# Autodesk Inventor assembly: battery_pack_16s.ipt
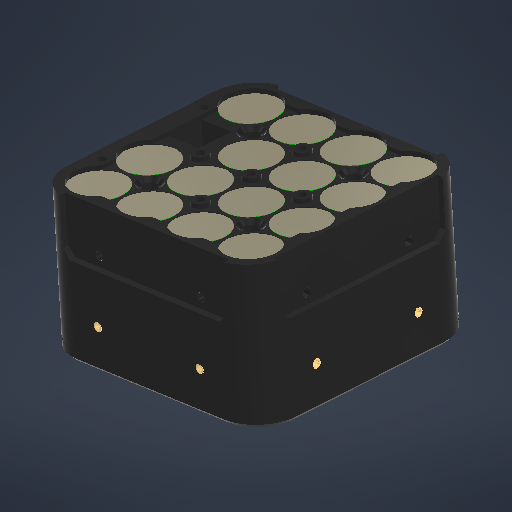
[picture p0: Inventor's stored thumbnail of the model, 512x512]
Saved by Autodesk Inventor 2026.1 (Build 301233000, 233)
## iProperties
Created: 2026-03-12
Part Number: battery_pack_16s.ipt
Document SubType Name: Assembly
Designer: aaron
Author: aaron
## Documents named in this file (6)
- D:\work\loopandpixel\openworkoutsystem\cad\v5\battery_pack_16s.ipt.iam
- D:\work\loopandpixel\openworkoutsystem\cad\v5\battery_26650_lifepo4.ipt
- D:\work\loopandpixel\openworkoutsystem\cad\v5\battery_pack_16s_front.ipt
- D:\work\loopandpixel\openworkoutsystem\cad\v5\battery_pack_cover_rear.ipt
- C:\Users\aaron\OneDrive\Documents\Inventor\Content Center Files\R2026\en-US\IS 6761\IS 6761 - M3 x 8 - 0.5.ipt
- D:\work\loopandpixel\openworkoutsystem\cad\v5\ruthex_RX-M3x5_7\ruthex_RX-M3x5_7\ruthex_RX-M3x5_7.iam
## Components (27 placed, 5 different names)
1. battery_pack_16s_front:1 — Insert:9, Mate:1, Flush:1, Flush:2, Insert:10, Insert:11, Insert:12, Insert:13, Insert:14, Insert:15
2. battery_pack_cover_rear:1 — Mate:1, Flush:1, Flush:2, Mate:2, Mate:3, Mate:4, Mate:5
3. IS 6761 M3 x 8:1 — Mate:2
4. IS 6761 M3 x 8:2 — Mate:3
5. IS 6761 M3 x 8:3 — Mate:4
6. IS 6761 M3 x 8:4 — Mate:5
7. ruthex_RX-M3x5_7:1 [sub-assembly] — Insert:11
8. ruthex_RX-M3x5_7:2 [sub-assembly] — Insert:10
9. ruthex_RX-M3x5_7:3 [sub-assembly] — Insert:12
10. ruthex_RX-M3x5_7:4 [sub-assembly] — Insert:13
11. ruthex_RX-M3x5_7:5 [sub-assembly] — Insert:14
12. ruthex_RX-M3x5_7:6 [sub-assembly] — Insert:15
13. battery_26650_lifepo4:1 — Insert:9
14. battery_26650_lifepo4:2
15. battery_26650_lifepo4:3
16. battery_26650_lifepo4:4
17. battery_26650_lifepo4:5
18. battery_26650_lifepo4:6
19. battery_26650_lifepo4:7
20. battery_26650_lifepo4:8
21. battery_26650_lifepo4:10
22. battery_26650_lifepo4:11
23. battery_26650_lifepo4:12
24. battery_26650_lifepo4:13
25. battery_26650_lifepo4:14
26. battery_26650_lifepo4:15
27. battery_26650_lifepo4:16
## Component patterns: (16 elements, first: battery_26650_lifepo4:1)
## Relationships (14: Insert 7, Mate 5, Flush 2)
- Insert:9: battery_pack_16s_front:1 ↔ battery_26650_lifepo4:1
- Mate:1: battery_pack_16s_front:1 ↔ battery_pack_cover_rear:1
- Flush:1: battery_pack_16s_front:1 ↔ battery_pack_cover_rear:1
- Flush:2: battery_pack_16s_front:1 ↔ battery_pack_cover_rear:1
- Mate:2: battery_pack_cover_rear:1 ↔ IS 6761 M3 x 8:1
- Mate:3: battery_pack_cover_rear:1 ↔ IS 6761 M3 x 8:2
- Mate:4: battery_pack_cover_rear:1 ↔ IS 6761 M3 x 8:3
- Mate:5: battery_pack_cover_rear:1 ↔ IS 6761 M3 x 8:4
- Insert:10: battery_pack_16s_front:1 ↔ ruthex_RX-M3x5_7:2
- Insert:11: battery_pack_16s_front:1 ↔ ruthex_RX-M3x5_7:1
- Insert:12: battery_pack_16s_front:1 ↔ ruthex_RX-M3x5_7:3
- Insert:13: battery_pack_16s_front:1 ↔ ruthex_RX-M3x5_7:4
- Insert:14: battery_pack_16s_front:1 ↔ ruthex_RX-M3x5_7:5
- Insert:15: battery_pack_16s_front:1 ↔ ruthex_RX-M3x5_7:6
